# Autodesk Inventor assembly: Test Assembly
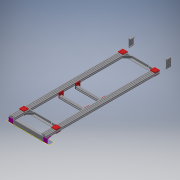
[picture p0: Inventor's stored thumbnail of the model, 180x180]
Saved by Autodesk Inventor 2016 SP2 (Build 200236200, 236)
## iProperties
Created: 2018-01-27
Part Number: Test Assembly
Document SubType Name: Assembly
Designer: CAD
Author: CAD
## Documents named in this file (9)
- C:\Users\CAD\Documents\GitHub\FIRST-ROBOTICS-2018-5436-CAD\Robot\Elevator\Test Assembly.iam
- C:\Users\CAD\Documents\GitHub\FIRST-ROBOTICS-2018-5436-CAD\Robot\Elevator\48 in 80-20 extrusion.ipt
- C:\Users\CAD\Documents\GitHub\FIRST-ROBOTICS-2018-5436-CAD\Robot\Elevator\80-20 extrusion rail.ipt
- C:\Users\CAD\Documents\GitHub\FIRST-ROBOTICS-2018-5436-CAD\Robot\Elevator\Bottom Elevator Bracket.ipt
- C:\Users\CAD\Documents\GitHub\FIRST-ROBOTICS-2018-5436-CAD\Robot\Elevator\10.75 in 80-20 extrusion.ipt
- C:\Users\CAD\Documents\GitHub\FIRST-ROBOTICS-2018-5436-CAD\Robot\Elevator\Triangle Bracket.ipt
- C:\Users\CAD\Documents\GitHub\FIRST-ROBOTICS-2018-5436-CAD\Robot\Elevator\11.25 in L.ipt
- C:\Users\CAD\Documents\GitHub\FIRST-ROBOTICS-2018-5436-CAD\Robot\Elevator\Upper Bracket of Elevator.ipt
- C:\Users\CAD\Documents\GitHub\FIRST-ROBOTICS-2018-5436-CAD\Robot\Elevator\Cross 2 x 1 beam on bottom of elevator.ipt
## Components (29 placed, 8 different names)
1. 48 in 80-20 extrusion:1 — Flush:1, Flush:3, Flush:5, Mate:16, Flush:12, Mate:26, Mate:27, Mate:70, Mate:71
2. 48 in 80-20 extrusion:2 — Flush:1, Mate:2, Mate:3, Mate:4, Mate:5, Flush:2, Mate:8, Mate:9, Mate:10, Mate:11, Flush:8, Flush:11, Mate:34, Mate:35, Mate:44, Mate:45, Mate:50, Mate:51, Mate:52, Mate:61, Mate:62, Flush:21
3. 48 in 80-20 extrusion:3 — Flush:5, Flush:6, Mate:19, Flush:11, Flush:13, Flush:14, Mate:39, Mate:40, Mate:46, Mate:47, Mate:53, Mate:54, Mate:58, Mate:59, Mate:60, Mate:67
4. 48 in 80-20 extrusion:4 — Flush:6, Mate:17, Mate:18, Mate:20, Mate:21, Flush:9, Flush:10, Flush:12, Mate:22, Mate:23, Mate:24, Mate:25, Mate:28, Mate:29, Flush:16, Mate:68, Mate:69
5. 80-20 extrusion rail:1 — Mate:2, Mate:3, Flush:2, Mate:6
6. 80-20 extrusion rail:2 — Mate:8, Mate:9, Flush:7, Mate:16
7. 80-20 extrusion rail:3 — Mate:10, Mate:11, Flush:8
8. 80-20 extrusion rail:4 — Mate:4, Mate:5, Flush:3, Mate:6, Flush:7
9. 80-20 extrusion rail:5 — Mate:17, Mate:18, Mate:19, Flush:9
10. 80-20 extrusion rail:8 — Mate:20, Mate:21, Flush:10
11. 80-20 extrusion rail:9 — Mate:24, Mate:25, Flush:14
12. 80-20 extrusion rail:10 — Mate:22, Mate:23, Flush:13
13. Bottom Elevator Bracket:1 — Mate:26, Mate:27, Flush:15, Angle:3, Mate:72
14. Bottom Elevator Bracket:2 — Mate:28, Mate:29, Flush:15, Flush:16, Mate:38, Flush:23, Flush:24
15. 80-20 extrusion rail:11 — Angle:2, Mate:39, Mate:40, Flush:17, Mate:41, Angle:4
16. 80-20 extrusion rail:12 — Mate:34, Mate:35, Angle:2, Flush:17, Mate:42, Mate:43, Mate:65
17. 10.75 in 80-20 extrusion:1 — Mate:41, Mate:42, Mate:43, Angle:4, Mate:66
18. Triangle Bracket:1 — Mate:44, Mate:45, Flush:18
19. Triangle Bracket:2 — Mate:46, Mate:47, Flush:18, Mate:48, Mate:49, Mate:67
20. 11.25 in L:1 — Mate:48, Mate:49, Mate:50
21. Triangle Bracket:3 — Mate:51, Mate:52, Mate:57, Flush:21
22. Triangle Bracket:4 — Mate:53, Mate:54, Mate:55, Mate:56
23. 11.25 in L:2 — Mate:55, Mate:56, Mate:57, Mate:58, Mate:65
24. 10.75 in 80-20 extrusion:2 — Mate:63, Mate:64, Angle:5, Mate:66
25. 80-20 extrusion rail:13 — Mate:59, Mate:60, Flush:19, Mate:63
26. 80-20 extrusion rail:14 — Mate:61, Mate:62, Flush:19, Mate:64, Angle:5
27. Upper Bracket of Elevator:1 — Mate:70, Mate:71, Flush:22
28. Upper Bracket of Elevator:2 — Mate:68, Mate:69, Flush:22
29. Cross 2 x 1 beam on bottom of elevator:1 — Flush:23, Mate:72, Flush:24
## Relationships (86: Mate 60, Flush 22, Angle 4)
- Flush:1: 48 in 80-20 extrusion:1 ↔ 48 in 80-20 extrusion:2
- Mate:2: 48 in 80-20 extrusion:2 ↔ 80-20 extrusion rail:1
- Mate:3: 48 in 80-20 extrusion:2 ↔ 80-20 extrusion rail:1
- Mate:4: 48 in 80-20 extrusion:2 ↔ 80-20 extrusion rail:4
- Mate:5: 48 in 80-20 extrusion:2 ↔ 80-20 extrusion rail:4
- Flush:2 (101.6 mm): 48 in 80-20 extrusion:2 ↔ 80-20 extrusion rail:1
- Flush:3: 48 in 80-20 extrusion:1 ↔ 80-20 extrusion rail:4
- Mate:6 (136.7282 mm): 80-20 extrusion rail:1 ↔ 80-20 extrusion rail:4
- Flush:5: 48 in 80-20 extrusion:1 ↔ 48 in 80-20 extrusion:3
- Flush:6: 48 in 80-20 extrusion:3 ↔ 48 in 80-20 extrusion:4
- Mate:8: 48 in 80-20 extrusion:2 ↔ 80-20 extrusion rail:2
- Mate:9: 48 in 80-20 extrusion:2 ↔ 80-20 extrusion rail:2
- Flush:7: 80-20 extrusion rail:2 ↔ 80-20 extrusion rail:4
- Mate:10: 48 in 80-20 extrusion:2 ↔ 80-20 extrusion rail:3
- Mate:11: 48 in 80-20 extrusion:2 ↔ 80-20 extrusion rail:3
- Flush:8 (101.6 mm): 48 in 80-20 extrusion:2 ↔ 80-20 extrusion rail:3
- Mate:16: 48 in 80-20 extrusion:1 ↔ 80-20 extrusion rail:2
- Mate:17: 48 in 80-20 extrusion:4 ↔ 80-20 extrusion rail:5
- Mate:18: 48 in 80-20 extrusion:4 ↔ 80-20 extrusion rail:5
- Mate:19: 48 in 80-20 extrusion:3 ↔ 80-20 extrusion rail:5
- Mate:20: 48 in 80-20 extrusion:4 ↔ 80-20 extrusion rail:8
- Mate:21: 48 in 80-20 extrusion:4 ↔ 80-20 extrusion rail:8
- Flush:9: 48 in 80-20 extrusion:4 ↔ 80-20 extrusion rail:5
- Flush:10: 48 in 80-20 extrusion:4 ↔ 80-20 extrusion rail:8
- Flush:11: 48 in 80-20 extrusion:2 ↔ 48 in 80-20 extrusion:3
- Flush:12: 48 in 80-20 extrusion:1 ↔ 48 in 80-20 extrusion:4
- Mate:22: 48 in 80-20 extrusion:4 ↔ 80-20 extrusion rail:10
- Mate:23: 48 in 80-20 extrusion:4 ↔ 80-20 extrusion rail:10
- Flush:13 (101.6 mm): 48 in 80-20 extrusion:3 ↔ 80-20 extrusion rail:10
- Mate:24: 48 in 80-20 extrusion:4 ↔ 80-20 extrusion rail:9
- Mate:25: 48 in 80-20 extrusion:4 ↔ 80-20 extrusion rail:9
- Flush:14 (-101.6 mm): 48 in 80-20 extrusion:3 ↔ 80-20 extrusion rail:9
- Mate:26: 48 in 80-20 extrusion:1 ↔ Bottom Elevator Bracket:1
- Mate:27: 48 in 80-20 extrusion:1 ↔ Bottom Elevator Bracket:1
- Mate:28: 48 in 80-20 extrusion:4 ↔ Bottom Elevator Bracket:2
- Mate:29: 48 in 80-20 extrusion:4 ↔ Bottom Elevator Bracket:2
- Flush:15: Bottom Elevator Bracket:1 ↔ Bottom Elevator Bracket:2
- Flush:16: 48 in 80-20 extrusion:4 ↔ Bottom Elevator Bracket:2
- Mate:34: 48 in 80-20 extrusion:2 ↔ 80-20 extrusion rail:12
- Mate:35: 48 in 80-20 extrusion:2 ↔ 80-20 extrusion rail:12
- Angle:2 (0 deg): 80-20 extrusion rail:11 ↔ 80-20 extrusion rail:12
- Mate:38: Bottom Elevator Bracket:2
- Angle:3 (0 deg): Bottom Elevator Bracket:1
- Mate:39: 48 in 80-20 extrusion:3 ↔ 80-20 extrusion rail:11
- Mate:40: 48 in 80-20 extrusion:3 ↔ 80-20 extrusion rail:11
- Flush:17: 80-20 extrusion rail:11 ↔ 80-20 extrusion rail:12
- Mate:41: 80-20 extrusion rail:11 ↔ 10.75 in 80-20 extrusion:1
- Mate:42: 80-20 extrusion rail:12 ↔ 10.75 in 80-20 extrusion:1
- Mate:43: 80-20 extrusion rail:12 ↔ 10.75 in 80-20 extrusion:1
- Angle:4 (0 deg): 80-20 extrusion rail:11 ↔ 10.75 in 80-20 extrusion:1
- Mate:44: 48 in 80-20 extrusion:2 ↔ Triangle Bracket:1
- Mate:45: 48 in 80-20 extrusion:2 ↔ Triangle Bracket:1
- Mate:46: 48 in 80-20 extrusion:3 ↔ Triangle Bracket:2
- Mate:47: 48 in 80-20 extrusion:3 ↔ Triangle Bracket:2
- Flush:18: Triangle Bracket:1 ↔ Triangle Bracket:2
- Mate:48: Triangle Bracket:2 ↔ 11.25 in L:1
- Mate:49: Triangle Bracket:2 ↔ 11.25 in L:1
- Mate:50 (1.27 mm): 48 in 80-20 extrusion:2 ↔ 11.25 in L:1
- Mate:51: 48 in 80-20 extrusion:2 ↔ Triangle Bracket:3
- Mate:52: 48 in 80-20 extrusion:2 ↔ Triangle Bracket:3
- Mate:53: 48 in 80-20 extrusion:3 ↔ Triangle Bracket:4
- Mate:54: 48 in 80-20 extrusion:3 ↔ Triangle Bracket:4
- Mate:55: Triangle Bracket:4 ↔ 11.25 in L:2
- Mate:56: Triangle Bracket:4 ↔ 11.25 in L:2
- Mate:57: Triangle Bracket:3 ↔ 11.25 in L:2
- Mate:58 (1.27 mm): 48 in 80-20 extrusion:3 ↔ 11.25 in L:2
- Mate:59: 48 in 80-20 extrusion:3 ↔ 80-20 extrusion rail:13
- Mate:60: 48 in 80-20 extrusion:3 ↔ 80-20 extrusion rail:13
- Mate:61: 48 in 80-20 extrusion:2 ↔ 80-20 extrusion rail:14
- Mate:62: 48 in 80-20 extrusion:2 ↔ 80-20 extrusion rail:14
- Flush:19: 80-20 extrusion rail:13 ↔ 80-20 extrusion rail:14
- Mate:63: 10.75 in 80-20 extrusion:2 ↔ 80-20 extrusion rail:13
- Mate:64: 10.75 in 80-20 extrusion:2 ↔ 80-20 extrusion rail:14
- Flush:21 (107.95 mm): 48 in 80-20 extrusion:2 ↔ Triangle Bracket:3
- Mate:65: 80-20 extrusion rail:12 ↔ 11.25 in L:2
- Angle:5 (0 deg): 10.75 in 80-20 extrusion:2 ↔ 80-20 extrusion rail:14
- Mate:66 (152.4 mm): 10.75 in 80-20 extrusion:1 ↔ 10.75 in 80-20 extrusion:2
- Mate:67 (-60.325 mm): 48 in 80-20 extrusion:3 ↔ Triangle Bracket:2
- Mate:68: 48 in 80-20 extrusion:4 ↔ Upper Bracket of Elevator:2
- Mate:69: 48 in 80-20 extrusion:4 ↔ Upper Bracket of Elevator:2
- Mate:70: 48 in 80-20 extrusion:1 ↔ Upper Bracket of Elevator:1
- Mate:71: 48 in 80-20 extrusion:1 ↔ Upper Bracket of Elevator:1
- Flush:22: Upper Bracket of Elevator:1 ↔ Upper Bracket of Elevator:2
- Flush:23: Bottom Elevator Bracket:2 ↔ Cross 2 x 1 beam on bottom of elevator:1
- Mate:72: Bottom Elevator Bracket:1 ↔ Cross 2 x 1 beam on bottom of elevator:1
- Flush:24: Bottom Elevator Bracket:2 ↔ Cross 2 x 1 beam on bottom of elevator:1
